# Autodesk Inventor assembly: Test rampy
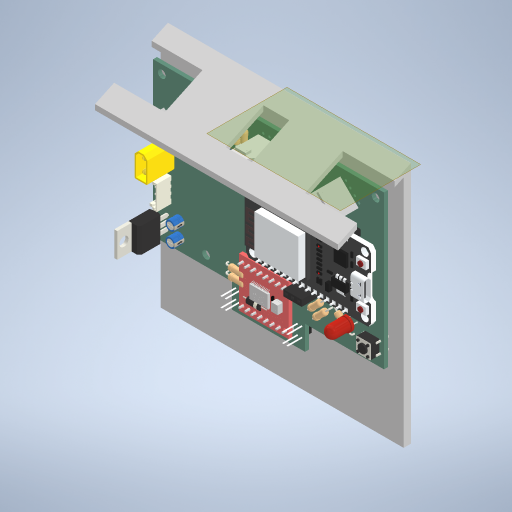
[picture p0: Inventor's stored thumbnail of the model, 512x512]
Saved by Autodesk Inventor 2024 (Build 280153000, 153)
## iProperties
Created: 2023-09-07
Part Number: Test rampy
Document SubType Name: Assembly
Designer: jaryj
Author: jaryj
## Documents named in this file (3)
- C:\Users\42060\Desktop\ŠKOLA\Mini sumo\RoboCop\- 3D -\temporary\Test rampy.iam
- C:\Users\42060\Desktop\ŠKOLA\Mini sumo\RoboCop\- 3D -\temporary\sumec\sumec.iam
- C:\Users\42060\Desktop\ŠKOLA\Mini sumo\RoboCop\- 3D -\temporary\Test rampy.ipt
## Components (2 placed, 2 different names)
1. sumec:1 [sub-assembly] — Stejný směr:1, Proti sobě:1, Proti sobě:2
2. Test rampy:1 — Stejný směr:1, Proti sobě:1, Proti sobě:2
## Relationships (3: Mate 2, Flush 1)
- Stejný směr:1 [Flush] (2.5 mm): sumec:1 ↔ Test rampy:1
- Proti sobě:1 [Mate] (4 mm): sumec:1 ↔ Test rampy:1
- Proti sobě:2 [Mate] (10.5 mm): sumec:1 ↔ Test rampy:1
